# Autodesk Inventor assembly: Refined functioning swerve drive
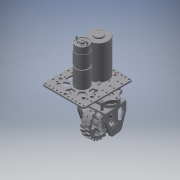
[picture p0: Inventor's stored thumbnail of the model, 180x180]
Saved by Autodesk Inventor 2019 (Build 230136000, 136)
## iProperties
Created: 2019-01-14
Part Number: Refined functioning swerve drive
Document SubType Name: Assembly
Designer: josh
Author: josh
## Documents named in this file (7)
- D:\Synthesis Robots\Epsilon\Refined functioning swerve drive.iam
- D:\Synthesis Robots\Epsilon\Functioning swerve drive sub-assemblies\Functioning swerve drive (casing).iam
- D:\Synthesis Robots\Epsilon\Functioning swerve drive sub-assemblies\Functioning swerve drive (adjacent shaft axel).iam
- D:\Synthesis Robots\Epsilon\Functioning swerve drive sub-assemblies\Functioning swerve drive (shaft axel).iam
- D:\Synthesis Robots\Epsilon\Functioning swerve drive sub-assemblies\Functioning Swerve drive (motor steering shaft).iam
- D:\Synthesis Robots\Epsilon\Swerve drive parts\Motor Mount Plate Rev 2.ipt
- D:\Synthesis Robots\Epsilon\Functioning swerve drive sub-assemblies\CIM motor and shaft.iam
## Components (6 placed, 6 different names)
1. Motor Mount Plate Rev 2:1 — Mate:23, Mate:24, Rotational:5, Mate:29, Mate:30, Mate:31
2. Functioning swerve drive (casing):1 [sub-assembly] — Mate:26, Rotational:6, Mate:27, Mate:28, Rotational:7
3. Functioning swerve drive (adjacent shaft axel):1 [sub-assembly] — Mate:27, Mate:28, Rotation:3
4. Functioning swerve drive (shaft axel):1 [sub-assembly] — Mate:26, Rotational:6, Rotation:3
5. Functioning Swerve drive (motor steering shaft):1 [sub-assembly] — Rotational:5
6. CIM motor and shaft:1 [sub-assembly] — Mate:29, Mate:30, Mate:31, Rotational:7
## Relationships (12: Mate 8, RevoluteJoint 3, RelateRotation 1)
- Mate:23: Motor Mount Plate Rev 2:1
- Mate:24: Motor Mount Plate Rev 2:1
- Rotational:5 [RevoluteJoint] (-2.54 mm): Motor Mount Plate Rev 2:1 ↔ Functioning Swerve drive (motor steering shaft):1
- Mate:26: Functioning swerve drive (casing):1 ↔ Functioning swerve drive (shaft axel):1
- Rotational:6 [RevoluteJoint]: Functioning swerve drive (casing):1 ↔ Functioning swerve drive (shaft axel):1
- Mate:27: Functioning swerve drive (casing):1 ↔ Functioning swerve drive (adjacent shaft axel):1
- Mate:28: Functioning swerve drive (casing):1 ↔ Functioning swerve drive (adjacent shaft axel):1
- Rotation:3 [RelateRotation] (0.5 ul): Functioning swerve drive (adjacent shaft axel):1 ↔ Functioning swerve drive (shaft axel):1
- Mate:29: Motor Mount Plate Rev 2:1 ↔ CIM motor and shaft:1
- Mate:30: Motor Mount Plate Rev 2:1 ↔ CIM motor and shaft:1
- Mate:31: Motor Mount Plate Rev 2:1 ↔ CIM motor and shaft:1
- Rotational:7 [RevoluteJoint]: Functioning swerve drive (casing):1 ↔ CIM motor and shaft:1
